# Autodesk Inventor assembly: étage
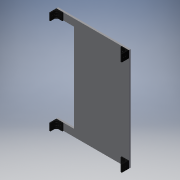
[picture p0: Inventor's stored thumbnail of the model, 180x180]
Saved by Autodesk Inventor 2019 (Build 230136000, 136)
## iProperties
Created: 2019-03-31
Part Number: étage
Document SubType Name: Assembly
Designer: franc
Author: franc
## Documents named in this file (3)
- C:\Users\franc\Desktop\EsialRobotik\Mecanique\2019\robot\étage.iam
- C:\Users\franc\Desktop\EsialRobotik\Mecanique\composants\Profile\equerreEtage.ipt
- C:\Users\franc\Desktop\EsialRobotik\Mecanique\2019\robot\étage.ipt
## Components (5 placed, 2 different names)
1. equerreEtage:1 — Placage:4, Affleurement:7, Affleurement:8
2. equerreEtage:2 — Placage:3, Affleurement:5, Affleurement:6
3. equerreEtage:3 — Placage:2, Affleurement:1, Affleurement:2
4. equerreEtage:4 — Placage:1, Affleurement:3, Affleurement:4
5. étage:1 — Placage:1, Placage:2, Placage:3, Placage:4, Affleurement:1, Affleurement:2, Affleurement:3, Affleurement:4, Affleurement:5, Affleurement:6, Affleurement:7, Affleurement:8
## Relationships (12: Flush 8, Mate 4)
- Placage:1 [Mate]: equerreEtage:4 ↔ étage:1
- Placage:2 [Mate]: equerreEtage:3 ↔ étage:1
- Placage:3 [Mate]: equerreEtage:2 ↔ étage:1
- Placage:4 [Mate]: equerreEtage:1 ↔ étage:1
- Affleurement:1 [Flush]: equerreEtage:3 ↔ étage:1
- Affleurement:2 [Flush]: equerreEtage:3 ↔ étage:1
- Affleurement:3 [Flush]: equerreEtage:4 ↔ étage:1
- Affleurement:4 [Flush]: equerreEtage:4 ↔ étage:1
- Affleurement:5 [Flush]: equerreEtage:2 ↔ étage:1
- Affleurement:6 [Flush]: equerreEtage:2 ↔ étage:1
- Affleurement:7 [Flush]: equerreEtage:1 ↔ étage:1
- Affleurement:8 [Flush]: equerreEtage:1 ↔ étage:1
